# Autodesk Inventor assembly: ExtruderP1
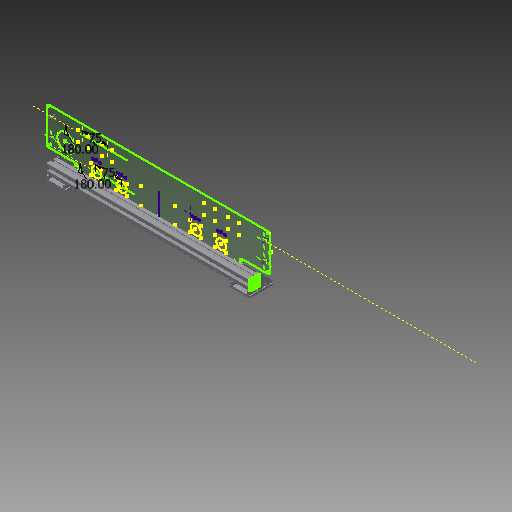
[picture p0: Inventor's stored thumbnail of the model, 512x512]
Saved by Autodesk Inventor 2017 (Build 210142000, 142)
## iProperties
Created: 2016-08-05
Part Number: ExtruderP1
Document SubType Name: Assembly
Designer: User
Author: User
## Documents named in this file (12)
- C:\All INVENTOR\SL-Inventor\SL-Beast 3D Printer\ExtruderP1.iam
- C:\All INVENTOR\SL-Inventor\SL-Beast 3D Printer\3030 600mm_CPY_CPY.ipt
- C:\All INVENTOR\SL-Inventor\SL-Beast 3D Printer\Y-Motor-Brace_MIR.ipt
- C:\All INVENTOR\SL-Inventor\SL-Beast 3D Printer\Y-Motor-Mount Top.ipt
- C:\All INVENTOR\SL-Inventor\SL-Beast 3D Printer\Y-Motor-Brace_MIR_MIR.ipt
- C:\All INVENTOR\SL-Inventor\SL-Beast 3D Printer\Y-Motor-Mount Top_MIR.ipt
- C:\All INVENTOR\SL-Inventor\SL-Beast 3D Printer\ExtruderPanel.iam
- C:\All INVENTOR\SL-Inventor\SL-Beast 3D Printer\en-US\ANSI B18.3.1M(6)\ANSI B18.3.1M - M3x0.5 x 16(1).ipt
- C:\All INVENTOR\SL-Inventor\SL-Beast 3D Printer\en-US\ANSI B18.3.1M(6)\ANSI B18.3.1M - M4x0.7 x 25(1).ipt
- C:\All INVENTOR\SL-Inventor\SL-Beast 3D Printer\M5 Tee Nut-Generic.ipt
- C:\All INVENTOR\SL-Inventor\SL-Beast 3D Printer\en-US\CSN EN 24 036\CSN EN 24 036 - M3.ipt
- C:\All INVENTOR\SL-Inventor\SL-Beast 3D Printer\M5 Tee Nut-Generic_MIR.ipt
## Components (24 placed, 11 different names)
1. 3030 600mm_CPY_CPY:1
2. Y-Motor-Mount Top:1
3. Y-Motor-Brace_MIR_MIR:1
4. Y-Motor-Brace_MIR_MIR:2
5. Y-Motor-Mount Top_MIR:1
6. ExtruderPanel:1 [sub-assembly]
7. Forged Socket Head Cap Screw - Metric M3x0.5 x 16:2
8. CSN EN 24036 M3:2
9. Forged Socket Head Cap Screw - Metric M3x0.5 x 16:1
10. CSN EN 24036 M3:1
11. Forged Socket Head Cap Screw - Metric M4x0.7 x 25:1
12. Forged Socket Head Cap Screw - Metric M4x0.7 x 25:2
13. M5 Tee Nut-Generic:2
14. M5 Tee Nut-Generic:1
15. Forged Socket Head Cap Screw - Metric M3x0.5 x 16:3
16. CSN EN 24036 M3:3
17. M5 Tee Nut-Generic_MIR:1
18. Forged Socket Head Cap Screw - Metric M4x0.7 x 25:3
19. Forged Socket Head Cap Screw - Metric M3x0.5 x 16:4
20. CSN EN 24036 M3:4
21. Forged Socket Head Cap Screw - Metric M4x0.7 x 25:4
22. M5 Tee Nut-Generic_MIR:2
23. Y-Motor-Brace_MIR:1
24. Y-Motor-Brace_MIR:2
## Component patterns: (2 elements, first: Y-Motor-Brace_MIR:1)
## Relationships (31: Mate 20, Insert 8, Flush 3)
- [Flush]: 3030 600mm_CPY_CPY:1 ↔ ExtruderPanel:1
- [Mate]: 3030 600mm_CPY_CPY:1 ↔ Y-Motor-Brace_MIR:1
- [Mate]: 3030 600mm_CPY_CPY:1 ↔ Y-Motor-Brace_MIR:1
- [Mate]: Y-Motor-Mount Top:1 ↔ Y-Motor-Brace_MIR:1
- [Mate]: Y-Motor-Mount Top:1 ↔ Y-Motor-Brace_MIR:1
- [Flush]: Y-Motor-Mount Top:1 ↔ Y-Motor-Brace_MIR:1
- [Flush]: Y-Motor-Brace_MIR_MIR:1 ↔ Y-Motor-Mount Top_MIR:1
- [Mate]: Y-Motor-Brace_MIR_MIR:1 ↔ Y-Motor-Mount Top_MIR:1
- [Mate]: Y-Motor-Brace_MIR_MIR:1 ↔ Y-Motor-Mount Top_MIR:1
- [Insert]: Y-Motor-Mount Top:1 ↔ Forged Socket Head Cap Screw - Metric M3x0.5 x 16:1
- [Insert]: Y-Motor-Mount Top:1 ↔ Forged Socket Head Cap Screw - Metric M3x0.5 x 16:2
- [Insert]: Y-Motor-Mount Top:1 ↔ Forged Socket Head Cap Screw - Metric M4x0.7 x 25:1
- [Insert]: Y-Motor-Mount Top:1 ↔ Forged Socket Head Cap Screw - Metric M4x0.7 x 25:2
- [Mate]: Forged Socket Head Cap Screw - Metric M4x0.7 x 25:1 ↔ M5 Tee Nut-Generic:1
- [Mate]: 3030 600mm_CPY_CPY:1 ↔ M5 Tee Nut-Generic:1
- [Mate]: Forged Socket Head Cap Screw - Metric M4x0.7 x 25:2 ↔ M5 Tee Nut-Generic:2
- [Mate]: 3030 600mm_CPY_CPY:1 ↔ M5 Tee Nut-Generic:2
- [Mate]: Forged Socket Head Cap Screw - Metric M3x0.5 x 16:1 ↔ CSN EN 24036 M3:1
- [Mate]: CSN EN 24036 M3:1 ↔ Y-Motor-Brace_MIR:1
- [Mate]: Forged Socket Head Cap Screw - Metric M3x0.5 x 16:2 ↔ CSN EN 24036 M3:2
- [Mate]: CSN EN 24036 M3:2 ↔ Y-Motor-Brace_MIR:2
- [Insert]: Y-Motor-Mount Top_MIR:1 ↔ Forged Socket Head Cap Screw - Metric M3x0.5 x 16:3
- [Insert]: Y-Motor-Mount Top_MIR:1 ↔ Forged Socket Head Cap Screw - Metric M3x0.5 x 16:4
- [Insert]: Y-Motor-Mount Top_MIR:1 ↔ Forged Socket Head Cap Screw - Metric M4x0.7 x 25:3
- [Insert]: Y-Motor-Mount Top_MIR:1 ↔ Forged Socket Head Cap Screw - Metric M4x0.7 x 25:4
- [Mate]: M5 Tee Nut-Generic_MIR:1 ↔ Forged Socket Head Cap Screw - Metric M4x0.7 x 25:3
- [Mate]: Forged Socket Head Cap Screw - Metric M4x0.7 x 25:4 ↔ M5 Tee Nut-Generic_MIR:2
- [Mate]: Y-Motor-Brace_MIR_MIR:1 ↔ CSN EN 24036 M3:3
- [Mate]: Forged Socket Head Cap Screw - Metric M3x0.5 x 16:3 ↔ CSN EN 24036 M3:3
- [Mate]: Forged Socket Head Cap Screw - Metric M3x0.5 x 16:4 ↔ CSN EN 24036 M3:4
- [Mate]: Y-Motor-Brace_MIR_MIR:2 ↔ CSN EN 24036 M3:4
